# Autodesk Inventor assembly: Rad_Axe_Gummi
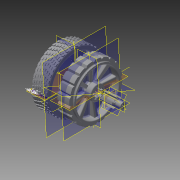
[picture p0: Inventor's stored thumbnail of the model, 180x180]
Saved by Autodesk Inventor 2015 (Build 190159000, 159)
## iProperties
Created: 2019-03-12
Part Number: Rad_Axe_Gummi
Document SubType Name: Assembly
Designer: Boris
Author: Boris
## Documents named in this file (4)
- D:\Wisag Hiserv\HiSERV Smart Drive\WorkOrder\3D - Teile\Rad_Axe_GummiVorne.iam
- D:\Wisag Hiserv\HiSERV Smart Drive\WorkOrder\3D - Teile\Rad.ipt
- D:\Wisag Hiserv\HiSERV Smart Drive\WorkOrder\3D - Teile\RadAxeVorne.ipt
- D:\Wisag Hiserv\HiSERV Smart Drive\WorkOrder\3D - Teile\RadGummi.ipt
## Components (3 placed, 3 different names)
1. Rad:1 — Einfügen:1, Einfügen:2
2. RadAxeVorne:1 — Einfügen:2
3. RadGummi:1 — Einfügen:1
## Relationships (2: Insert 2)
- Einfügen:1 [Insert] (30 mm): Rad:1 ↔ RadGummi:1
- Einfügen:2 [Insert] (10 mm): Rad:1 ↔ RadAxeVorne:1
